# Autodesk Inventor assembly: Estructura matriz centelladora
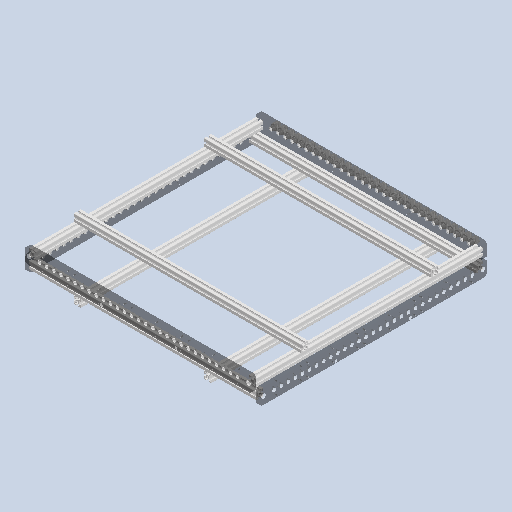
[picture p0: Inventor's stored thumbnail of the model, 512x512]
Saved by Autodesk Inventor 2024.2 (Build 282272000, 272)
## iProperties
Created: 2024-08-23
Part Number: Estructura matriz centelladora
Document SubType Name: Assembly
Designer: ja.restrepo1
Author: ja.restrepo1
## Documents named in this file (9)
- I:\MICROMECANICA\ALTAS ENERGIAS\Deteccion de Muones\Detectores centelladores\Partes Detector Centellador\SE Matriz Centelladora DC\SSE Estructura Centelladoras 20x20 DC\SSE estructura matriz centelladora.iam
- I:\MICROMECANICA\ALTAS ENERGIAS\Deteccion de Muones\Detectores\Detectores centelladores\Partes Detectores centelladores\PARTES DC\Perfileria 20x20 DC\Perfil 20X20 T.ipt
- I:\MICROMECANICA\ALTAS ENERGIAS\Deteccion de Muones\Detectores centelladores\Partes Detector Centellador\SE Matriz Centelladora DC\SSE Estructura Centelladoras 20x20 DC\Perfil 20X20 T\Perfil 20X20 T-620BCAM5.ipt
- I:\MICROMECANICA\ALTAS ENERGIAS\Deteccion de Muones\Detectores centelladores\Partes Detector Centellador\SE Matriz Centelladora DC\SSE Estructura Centelladoras 20x20 DC\Perfil 20X20 T\Perfil 20X20 T-620M5.ipt
- I:\MICROMECANICA\ALTAS ENERGIAS\Deteccion de Muones\Detectores centelladores\Partes Detector Centellador\SE Matriz Centelladora DC\SSE Estructura Centelladoras 20x20 DC\Perfil 20X20 T\Perfil 20X20 T-620Ø5.ipt
- I:\MICROMECANICA\ALTAS ENERGIAS\Deteccion de Muones\Detectores centelladores\Partes Detector Centellador\SE Matriz Centelladora DC\Extremos centella DC\Extremo centella\Extremo centella Soporte IC.ipt
- I:\MICROMECANICA\ALTAS ENERGIAS\Deteccion de Muones\Detectores centelladores\Partes Detectores centelladores\PARTES DC\Extremos centella DC\Extremo centella.ipt
- I:\MICROMECANICA\ALTAS ENERGIAS\Deteccion de Muones\Detectores centelladores\Partes Detector Centellador\SE Matriz Centelladora DC\Extremos centella DC\Extremo centella\Extremo centella entrada fibra OP.ipt
- I:\MICROMECANICA\ALTAS ENERGIAS\Deteccion de Muones\Detectores centelladores\Partes Detector Centellador\SE Matriz Centelladora DC\Ferula Fiber Op\SSE Ferula FO DC.iam
## Components (70 placed, 6 different names)
1. Perfil 20X20 T-620BCAM5:1 — Nivelación:2, Nivelación:3, Coincidencia:2, Nivelación:10, Coincidencia:4, Nivelación:19, Coincidencia:10, Nivelación:22, Coincidencia:13, Coincidencia:16, Coincidencia:17, Coincidencia:21, Coincidencia:23
2. Perfil 20X20 T-620BCAM5:2 — Nivelación:1, Nivelación:3, Nivelación:8, Nivelación:9, Coincidencia:3, Coincidencia:4, Coincidencia:15, Coincidencia:22
3. Perfil 20X20 T-620M5:3 — Nivelación:6, Nivelación:7, Nivelación:8, Coincidencia:3, Nivelación:10, Nivelación:24, Coincidencia:14, Coincidencia:18, Coincidencia:24, Coincidencia:26
4. Perfil 20X20 T-620M5:4 — Nivelación:5, Nivelación:7, Nivelación:9, Coincidencia:11, Coincidencia:19, Coincidencia:20, Coincidencia:25
5. Perfil 20X20 T-620Ø5:5 — Nivelación:19, Coincidencia:9, Nivelación:20, Nivelación:21, Coincidencia:10, Nivelación:22, Coincidencia:11
6. Perfil 20X20 T-620Ø5:6 — Coincidencia:9, Nivelación:20, Nivelación:21
7. Perfil 20X20 T-620Ø5:7 — Nivelación:23, Coincidencia:12, Nivelación:24, Nivelación:25, Coincidencia:13, Coincidencia:14
8. Perfil 20X20 T-620Ø5:8 — Nivelación:23, Coincidencia:12, Nivelación:25
9. Extremo centella Soporte IC:1 — Coincidencia:15, Coincidencia:16, Coincidencia:17
10. Extremo centella Soporte IC:2 — Coincidencia:18, Coincidencia:19, Coincidencia:20
11. Extremo centella entrada fibra OP:3 — Coincidencia:21, Coincidencia:22, Coincidencia:23, Coincidencia:27, Nivelación:26
12. Extremo centella entrada fibra OP:4 — Coincidencia:24, Coincidencia:25, Coincidencia:26, Coincidencia:28, Nivelación:27
13. SSE Ferula FO DC:1 [sub-assembly] — Coincidencia:27, Nivelación:26
14. SSE Ferula FO DC:2 [sub-assembly]
15. SSE Ferula FO DC:3 [sub-assembly]
16. SSE Ferula FO DC:4 [sub-assembly]
17. SSE Ferula FO DC:5 [sub-assembly]
18. SSE Ferula FO DC:6 [sub-assembly]
19. SSE Ferula FO DC:7 [sub-assembly]
20. SSE Ferula FO DC:8 [sub-assembly]
21. SSE Ferula FO DC:9 [sub-assembly]
22. SSE Ferula FO DC:10 [sub-assembly]
23. SSE Ferula FO DC:11 [sub-assembly]
24. SSE Ferula FO DC:12 [sub-assembly]
25. SSE Ferula FO DC:13 [sub-assembly]
26. SSE Ferula FO DC:14 [sub-assembly]
27. SSE Ferula FO DC:15 [sub-assembly]
28. SSE Ferula FO DC:16 [sub-assembly]
29. SSE Ferula FO DC:17 [sub-assembly]
30. SSE Ferula FO DC:18 [sub-assembly]
31. SSE Ferula FO DC:19 [sub-assembly]
32. SSE Ferula FO DC:20 [sub-assembly]
33. SSE Ferula FO DC:21 [sub-assembly]
34. SSE Ferula FO DC:22 [sub-assembly]
35. SSE Ferula FO DC:23 [sub-assembly]
36. SSE Ferula FO DC:24 [sub-assembly]
37. SSE Ferula FO DC:25 [sub-assembly]
38. SSE Ferula FO DC:26 [sub-assembly]
39. SSE Ferula FO DC:27 [sub-assembly]
40. SSE Ferula FO DC:28 [sub-assembly]
41. SSE Ferula FO DC:29 [sub-assembly]
42. SSE Ferula FO DC:30 [sub-assembly] — Coincidencia:28, Nivelación:27
43. SSE Ferula FO DC:31 [sub-assembly]
44. SSE Ferula FO DC:32 [sub-assembly]
45. SSE Ferula FO DC:33 [sub-assembly]
46. SSE Ferula FO DC:34 [sub-assembly]
47. SSE Ferula FO DC:35 [sub-assembly]
48. SSE Ferula FO DC:36 [sub-assembly]
49. SSE Ferula FO DC:37 [sub-assembly]
50. SSE Ferula FO DC:38 [sub-assembly]
51. SSE Ferula FO DC:39 [sub-assembly]
52. SSE Ferula FO DC:40 [sub-assembly]
53. SSE Ferula FO DC:41 [sub-assembly]
54. SSE Ferula FO DC:42 [sub-assembly]
55. SSE Ferula FO DC:43 [sub-assembly]
56. SSE Ferula FO DC:44 [sub-assembly]
57. SSE Ferula FO DC:45 [sub-assembly]
58. SSE Ferula FO DC:46 [sub-assembly]
59. SSE Ferula FO DC:47 [sub-assembly]
60. SSE Ferula FO DC:48 [sub-assembly]
61. SSE Ferula FO DC:49 [sub-assembly]
62. SSE Ferula FO DC:50 [sub-assembly]
63. SSE Ferula FO DC:51 [sub-assembly]
64. SSE Ferula FO DC:52 [sub-assembly]
65. SSE Ferula FO DC:53 [sub-assembly]
66. SSE Ferula FO DC:54 [sub-assembly]
67. SSE Ferula FO DC:55 [sub-assembly]
68. SSE Ferula FO DC:56 [sub-assembly]
69. SSE Ferula FO DC:57 [sub-assembly]
70. SSE Ferula FO DC:58 [sub-assembly]
## Component patterns: Ferula Fibra Optica (29 elements), Ferula Fibra Optica1 (29 elements)
## Relationships (41: Mate 23, Flush 18)
- Nivelación:1 [Flush]: Perfil 20X20 T-620BCAM5:2
- Nivelación:2 [Flush]: Perfil 20X20 T-620BCAM5:1
- Nivelación:3 [Flush]: Perfil 20X20 T-620BCAM5:1 ↔ Perfil 20X20 T-620BCAM5:2
- Coincidencia:2 [Mate] (5 mm): Perfil 20X20 T-620BCAM5:1
- Nivelación:5 [Flush]: Perfil 20X20 T-620M5:4
- Nivelación:6 [Flush]: Perfil 20X20 T-620M5:3
- Nivelación:7 [Flush]: Perfil 20X20 T-620M5:3 ↔ Perfil 20X20 T-620M5:4
- Nivelación:8 [Flush]: Perfil 20X20 T-620BCAM5:2 ↔ Perfil 20X20 T-620M5:3
- Nivelación:9 [Flush]: Perfil 20X20 T-620BCAM5:2 ↔ Perfil 20X20 T-620M5:4
- Coincidencia:3 [Mate] (10 mm): Perfil 20X20 T-620BCAM5:2 ↔ Perfil 20X20 T-620M5:3
- Nivelación:10 [Flush]: Perfil 20X20 T-620BCAM5:1 ↔ Perfil 20X20 T-620M5:3
- Coincidencia:4 [Mate] (570 mm): Perfil 20X20 T-620BCAM5:1 ↔ Perfil 20X20 T-620BCAM5:2
- Nivelación:19 [Flush]: Perfil 20X20 T-620BCAM5:1 ↔ Perfil 20X20 T-620Ø5:5
- Coincidencia:9 [Mate] (330 mm): Perfil 20X20 T-620Ø5:5 ↔ Perfil 20X20 T-620Ø5:6
- Nivelación:20 [Flush]: Perfil 20X20 T-620Ø5:5 ↔ Perfil 20X20 T-620Ø5:6
- Nivelación:21 [Flush]: Perfil 20X20 T-620Ø5:5 ↔ Perfil 20X20 T-620Ø5:6
- Coincidencia:10 [Mate]: Perfil 20X20 T-620BCAM5:1 ↔ Perfil 20X20 T-620Ø5:5
- Nivelación:22 [Flush]: Perfil 20X20 T-620BCAM5:1 ↔ Perfil 20X20 T-620Ø5:5
- Coincidencia:11 [Mate] (100 mm): Perfil 20X20 T-620M5:4 ↔ Perfil 20X20 T-620Ø5:5
- Nivelación:23 [Flush]: Perfil 20X20 T-620Ø5:7 ↔ Perfil 20X20 T-620Ø5:8
- Coincidencia:12 [Mate] (330 mm): Perfil 20X20 T-620Ø5:7 ↔ Perfil 20X20 T-620Ø5:8
- Nivelación:24 [Flush]: Perfil 20X20 T-620M5:3 ↔ Perfil 20X20 T-620Ø5:7
- Nivelación:25 [Flush]: Perfil 20X20 T-620Ø5:7 ↔ Perfil 20X20 T-620Ø5:8
- Coincidencia:13 [Mate] (100 mm): Perfil 20X20 T-620BCAM5:1 ↔ Perfil 20X20 T-620Ø5:7
- Coincidencia:14 [Mate]: Perfil 20X20 T-620M5:3 ↔ Perfil 20X20 T-620Ø5:7
- Coincidencia:15 [Mate]: Perfil 20X20 T-620BCAM5:2 ↔ Extremo centella Soporte IC:1
- Coincidencia:16 [Mate]: Perfil 20X20 T-620BCAM5:1 ↔ Extremo centella Soporte IC:1
- Coincidencia:17 [Mate]: Perfil 20X20 T-620BCAM5:1 ↔ Extremo centella Soporte IC:1
- Coincidencia:18 [Mate]: Perfil 20X20 T-620M5:3 ↔ Extremo centella Soporte IC:2
- Coincidencia:19 [Mate]: Perfil 20X20 T-620M5:4 ↔ Extremo centella Soporte IC:2
- Coincidencia:20 [Mate]: Perfil 20X20 T-620M5:4 ↔ Extremo centella Soporte IC:2
- Coincidencia:21 [Mate]: Perfil 20X20 T-620BCAM5:1 ↔ Extremo centella entrada fibra OP:3
- Coincidencia:22 [Mate]: Perfil 20X20 T-620BCAM5:2 ↔ Extremo centella entrada fibra OP:3
- Coincidencia:23 [Mate]: Perfil 20X20 T-620BCAM5:1 ↔ Extremo centella entrada fibra OP:3
- Coincidencia:24 [Mate]: Perfil 20X20 T-620M5:3 ↔ Extremo centella entrada fibra OP:4
- Coincidencia:25 [Mate]: Perfil 20X20 T-620M5:4 ↔ Extremo centella entrada fibra OP:4
- Coincidencia:26 [Mate]: Perfil 20X20 T-620M5:3 ↔ Extremo centella entrada fibra OP:4
- Coincidencia:27 [Mate]: Extremo centella entrada fibra OP:3 ↔ SSE Ferula FO DC:1
- Nivelación:26 [Flush] (1.6 mm): Extremo centella entrada fibra OP:3 ↔ SSE Ferula FO DC:1
- Coincidencia:28 [Mate]: Extremo centella entrada fibra OP:4 ↔ SSE Ferula FO DC:30
- Nivelación:27 [Flush] (1.5 mm): Extremo centella entrada fibra OP:4 ↔ SSE Ferula FO DC:30
